# Autodesk Inventor assembly: narrow high rectangular -0
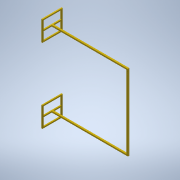
[picture p0: Inventor's stored thumbnail of the model, 180x180]
Saved by Autodesk Inventor 2021 (Build 250183000, 183)
## iProperties
Created: 2024-04-18
Part Number: narrow high rectangular -0
Document SubType Name: Assembly
Designer: Michal
Author: Michal
## Documents named in this file (7)
- C:\Users\Michal\Documents\GitHub\PNW_PhotoBoothFrame_3D\narrow high rectangular\narrow high rectangular -0.iam
- C:\Users\Michal\Documents\GitHub\PNW_PhotoBoothFrame_3D\narrow high rectangular\narrow high rectangular -0.1.iam
- C:\Users\Michal\Documents\GitHub\PNW_PhotoBoothFrame_3D\narrow high rectangular\narrow high rectangular -0.2.iam
- C:\Users\Michal\Documents\GitHub\PNW_PhotoBoothFrame_3D\narrow high rectangular\beam 30x30x2 -1.ipt
- C:\Users\Michal\Documents\GitHub\PNW_PhotoBoothFrame_3D\M8x15.ipt
- C:\Users\Michal\Documents\GitHub\PNW_PhotoBoothFrame_3D\narrow high rectangular\beam 30x30x2 -2.ipt
- C:\Users\Michal\Documents\GitHub\PNW_PhotoBoothFrame_3D\narrow high rectangular\beam 30x30x2 -3.ipt
## Components (9 placed, 6 different names)
1. narrow high rectangular -0.1:1 [sub-assembly] — Flush:1, Flush:2, Mate:1, Flush:3, Mate:2, Mate:3, Mate:5
2. narrow high rectangular -0.1:2 [sub-assembly] — Flush:1, Flush:2, Mate:10, Flush:4, Flush:5, Mate:11
3. narrow high rectangular -0.2:1 [sub-assembly] — Mate:12, Mate:13, Mate:14, Mate:15
4. narrow high rectangular -0.2:2 [sub-assembly] — Mate:7, Mate:8, Mate:9, Mate:17
5. beam 30x30x2 -1:1 — Mate:1, Flush:3, Mate:2, Mate:4, Mate:6, Mate:7, Mate:8, Mate:9
6. M8x15:1 — Mate:3, Mate:4
7. M8x15:2 — Mate:5, Mate:6
8. beam 30x30x2 -2:1 — Mate:10, Flush:4, Flush:5, Mate:11, Mate:12, Mate:13, Mate:14, Flush:6
9. beam 30x30x2 -3:1 — Flush:6, Mate:15, Mate:17
## Relationships (22: Mate 16, Flush 6)
- Flush:1: narrow high rectangular -0.1:1 ↔ narrow high rectangular -0.1:2
- Flush:2: narrow high rectangular -0.1:1 ↔ narrow high rectangular -0.1:2
- Mate:1: narrow high rectangular -0.1:1 ↔ beam 30x30x2 -1:1
- Flush:3: narrow high rectangular -0.1:1 ↔ beam 30x30x2 -1:1
- Mate:2: narrow high rectangular -0.1:1 ↔ beam 30x30x2 -1:1
- Mate:3: narrow high rectangular -0.1:1 ↔ M8x15:1
- Mate:4: beam 30x30x2 -1:1 ↔ M8x15:1
- Mate:5: narrow high rectangular -0.1:1 ↔ M8x15:2
- Mate:6: beam 30x30x2 -1:1 ↔ M8x15:2
- Mate:7: narrow high rectangular -0.2:2 ↔ beam 30x30x2 -1:1
- Mate:8: narrow high rectangular -0.2:2 ↔ beam 30x30x2 -1:1
- Mate:9: narrow high rectangular -0.2:2 ↔ beam 30x30x2 -1:1
- Mate:10: narrow high rectangular -0.1:2 ↔ beam 30x30x2 -2:1
- Flush:4: narrow high rectangular -0.1:2 ↔ beam 30x30x2 -2:1
- Flush:5: narrow high rectangular -0.1:2 ↔ beam 30x30x2 -2:1
- Mate:11: narrow high rectangular -0.1:2 ↔ beam 30x30x2 -2:1
- Mate:12: narrow high rectangular -0.2:1 ↔ beam 30x30x2 -2:1
- Mate:13: narrow high rectangular -0.2:1 ↔ beam 30x30x2 -2:1
- Mate:14: narrow high rectangular -0.2:1 ↔ beam 30x30x2 -2:1
- Flush:6: beam 30x30x2 -2:1 ↔ beam 30x30x2 -3:1
- Mate:15: narrow high rectangular -0.2:1 ↔ beam 30x30x2 -3:1
- Mate:17: narrow high rectangular -0.2:2 ↔ beam 30x30x2 -3:1
